# Autodesk Inventor assembly: joint4
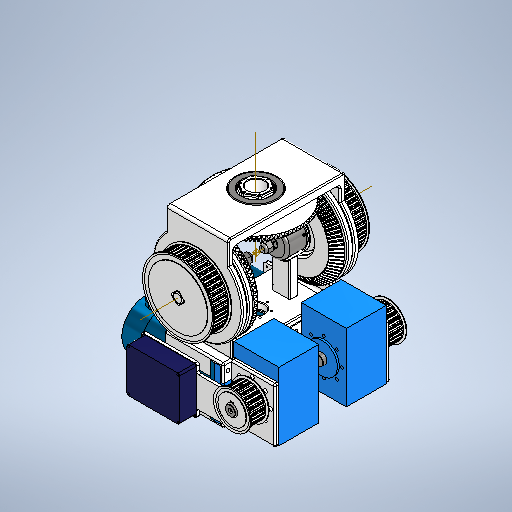
[picture p0: Inventor's stored thumbnail of the model, 512x512]
Saved by Autodesk Inventor 2025.3 (Build 293356030, 356C)
## iProperties
Created: 2025-08-31
Part Number: joint4
Document SubType Name: Assembly
Designer: MSI
Mass: 18656.6 g
Surface Area: 12044 cm^2
Volume: 7947.71 cm^3
Density: 2.34742 g/cm^3
Author: MSI
## Documents named in this file (14)
- C:\Users\MSI\Desktop\Project\3. 로봇팔\Robot Arm Model\Robot_Arm_6_v1\joint4.iam
- C:\Users\MSI\Desktop\Project\3. 로봇팔\Robot Arm Model\Robot_Arm_6_v1\encoder.ipt
- C:\Users\MSI\Desktop\Project\3. 로봇팔\Robot Arm Model\Robot_Arm_6_v1\encoder_supporter.ipt
- C:\Users\MSI\Desktop\Project\3. 로봇팔\Robot Arm Model\Robot_Arm_6_v1\joint4_frame.ipt
- C:\Users\MSI\Desktop\Project\3. 로봇팔\Robot Arm Model\Robot_Arm_6_v1\motor.iam
- C:\Users\MSI\Desktop\Project\3. 로봇팔\Robot Arm Model\Robot_Arm_6_v1\C-E6704ZZ_Autodesk_Inventor_2024_20250921\C-E6704ZZ.ipt
- C:\Users\MSI\Desktop\Project\3. 로봇팔\Robot Arm Model\Robot_Arm_6_v1\joint4_base.ipt
- C:\Users\MSI\Desktop\Project\3. 로봇팔\Robot Arm Model\Robot_Arm_6_v1\C-E6810ZZ_Autodesk_Inventor_2024_20250921\C-E6810ZZ.ipt
- C:\Users\MSI\Desktop\Project\3. 로봇팔\Robot Arm Model\Robot_Arm_6_v1\NTN_GS81110OuterRings\GS81110Outer Rings.ipt
- C:\Users\MSI\Desktop\Project\3. 로봇팔\Robot Arm Model\Robot_Arm_6_v1\joint4\디자인 액셀러레이터\베벨 기어1.iam
- C:\Users\MSI\Desktop\Project\3. 로봇팔\Robot Arm Model\Robot_Arm_6_v1\joint4\디자인 액셀러레이터\베벨 기어11.ipt
- C:\Users\MSI\Desktop\Project\3. 로봇팔\Robot Arm Model\Robot_Arm_6_v1\joint4_belt_pully2\driven_pulley.iam
- C:\Users\MSI\Desktop\Project\3. 로봇팔\Robot Arm Model\Robot_Arm_6_v1\joint4_belt_pully1\driving_pulley.iam
- C:\Users\MSI\Desktop\Project\3. 로봇팔\Robot Arm Model\Robot_Arm_6_v1\Robot_Arm_Parameter.xlsx
## Components (20 placed, 12 different names)
1. motor:1 [sub-assembly] — 삽입:1, 삽입:8, 삽입:10
2. joint4_base:1 — 삽입:1, 메이트:1, 메이트:2, 삽입:2, 삽입:3, 메이트:3, 메이트:4, 메이트:5
3. joint4_frame:1 — 삽입:5, 삽입:6, 메이트:7, 메이트:8, 삽입:12, 삽입:13, 삽입:14
4. encoder:1 — 삽입:7
5. encoder:2 — 삽입:4
6. encoder_supporter:1 — 메이트:5, 삽입:4
7. encoder_supporter:2 — 메이트:4, 삽입:7
8. C-E6704ZZ:1 — 삽입:6
9. C-E6704ZZ:2 — 삽입:5
10. C-E6704ZZ:3 — 삽입:3
11. C-E6704ZZ:4 — 삽입:2
12. C-E6810ZZ:1 — 삽입:14
13. GS81110Outer Rings:1 — 삽입:13
14. GS81110Outer Rings:2 — 삽입:12
15. 베벨 기어:1 [sub-assembly] — 메이트:1, 메이트:2, 메이트:6, 메이트:7, 삽입:11
16. 베벨 기어1:3 — 메이트:3, 메이트:6, 메이트:8, 삽입:9
17. driven_pulley:1 [sub-assembly] — 삽입:9
18. driving_pulley:1 [sub-assembly] — 삽입:8
19. driven_pulley:2 [sub-assembly] — 삽입:11
20. driving_pulley:2 [sub-assembly] — 삽입:10
## Relationships (22: Insert 14, Mate 8)
- 삽입:1 [Insert]: motor:1 ↔ joint4_base:1
- 메이트:1 [Mate]: joint4_base:1 ↔ 베벨 기어:1
- 메이트:2 [Mate]: joint4_base:1 ↔ 베벨 기어:1
- 삽입:2 [Insert]: joint4_base:1 ↔ C-E6704ZZ:4
- 삽입:3 [Insert]: joint4_base:1 ↔ C-E6704ZZ:3
- 메이트:3 [Mate]: joint4_base:1 ↔ 베벨 기어1:3
- 메이트:4 [Mate]: joint4_base:1 ↔ encoder_supporter:2
- 메이트:5 [Mate]: joint4_base:1 ↔ encoder_supporter:1
- 삽입:4 [Insert]: encoder:2 ↔ encoder_supporter:1
- 삽입:5 [Insert]: joint4_frame:1 ↔ C-E6704ZZ:2
- 삽입:6 [Insert]: joint4_frame:1 ↔ C-E6704ZZ:1
- 메이트:6 [Mate]: 베벨 기어:1 ↔ 베벨 기어1:3
- 삽입:7 [Insert]: encoder:1 ↔ encoder_supporter:2
- 메이트:7 [Mate]: joint4_frame:1 ↔ 베벨 기어:1
- 메이트:8 [Mate]: joint4_frame:1 ↔ 베벨 기어1:3
- 삽입:8 [Insert]: motor:1 ↔ driving_pulley:1
- 삽입:9 [Insert]: 베벨 기어1:3 ↔ driven_pulley:1
- 삽입:10 [Insert]: motor:1 ↔ driving_pulley:2
- 삽입:11 [Insert]: 베벨 기어:1 ↔ driven_pulley:2
- 삽입:12 [Insert]: joint4_frame:1 ↔ GS81110Outer Rings:2
- 삽입:13 [Insert]: joint4_frame:1 ↔ GS81110Outer Rings:1
- 삽입:14 [Insert] (1 mm): joint4_frame:1 ↔ C-E6810ZZ:1
## Named parameters: joint4_belt_centor = 157.367 mm, joint4_axis2_L = 58.803 mm, joint4_axis2_b1 = 35 mm, joint4_axis2_b2 = 10 mm, joint4_axis2_d = 18.17272 mm, joint4_miter_m = 2 mm, joint4_miter_a = 20 deg, joint4_miter_z = 79 mm, joint4_miter_b = 6.90139 mm, joint4_axis3_L = 23.5 mm, joint4_axis3_d1 = 30 mm, joint4_axis3_d2 = 50 mm, joint3_belt_centor = 157.367 mm, joint3_axis2_L = 16 mm, joint3_axis2_b1 = 10 mm, joint3_axis2_d = 18.1351 mm, joint3_planetary_m = 1.5 mm, joint3_planetary_a = 20 deg, joint3_planetary_np = 4 mm, joint3_sun_z = 18 mm, joint3_sun_b = 16.95546 mm, joint3_planet_z = 36 mm, joint3_planet_b = 16.95546 mm, joint3_ring_z = 90 mm, joint3_ring_b = 8.91686 mm, joint3_axis3_L = 10 mm, joint3_axis3_d = 28.08742 mm, joint3_miter_m = 5.5 mm, joint3_miter_a = 20 deg, joint3_miter_z = 28 mm, joint3_miter_b = 13.65957 mm, joint3_axis4_L = 23.5 mm, joint3_axis4_d1 = 30 mm, joint3_axis4_d2 = 50 mm
